# Autodesk Inventor assembly: servo_bracket
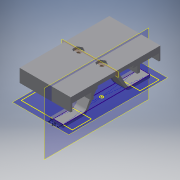
[picture p0: Inventor's stored thumbnail of the model, 180x180]
Saved by Autodesk Inventor 2018 (Build 220112000, 112)
## iProperties
Created: 2018-03-19
Part Number: servo_bracket
Document SubType Name: Assembly
Designer: erwin
Author: erwin
## Documents named in this file (3)
- D:\GitHub\SSJeVoisWheeledCargoShip\design\servo_bracket.iam
- D:\GitHub\SSJeVoisWheeledCargoShip\design\servo_bracket_lower_center_gravity.ipt
- D:\GitHub\SSJeVoisWheeledCargoShip\design\servo_bracket_holder.ipt
## Components (2 placed, 2 different names)
1. servo_bracket_lower_center_gravity:1 — Flush:1, Flush:4
2. servo_bracket_holder:1 — Flush:2, Flush:3, Flush:4
## Relationships (4: Flush 4)
- Flush:1 (22.8 mm): servo_bracket_lower_center_gravity:1
- Flush:2: servo_bracket_holder:1
- Flush:3: servo_bracket_holder:1
- Flush:4: servo_bracket_lower_center_gravity:1 ↔ servo_bracket_holder:1
